# Autodesk Inventor assembly: TelescopingArm_MIR1
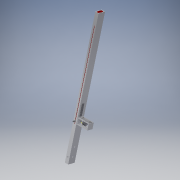
[picture p0: Inventor's stored thumbnail of the model, 180x180]
Saved by Autodesk Inventor 2016 SP1 (Build 200210100, 210)
## iProperties
Created: 2016-01-26
Part Number: TelescopingArm_MIR1
Document SubType Name: Assembly
Designer: steele
Mass: 2430.38 g
Surface Area: 5620.49 cm^2
Volume: 865.213 cm^3
Density: 2.80899 g/cm^3
Author: steele
## Documents named in this file (7)
- C:\snobotics\CAD-Development\robSteele\SnoBotics2016\TelescopeArm\TelescopingArm_MIR1.iam
- C:\snobotics\CAD-Development\robSteele\SnoBotics2016\TelescopeArm\OuterTube_MIR2.ipt
- C:\snobotics\CAD-Development\robSteele\SnoBotics2016\TelescopeArm\InnerTube_MIR2.ipt
- C:\snobotics\CAD-Development\robSteele\SnoBotics2016\2016-01-31-Lift\InnerTubeStopPost_MIR.ipt
- C:\snobotics\CAD-Development\robSteele\SnoBotics2016\2016-02-17-StopMechanism\StopMechanismAssembly_MIR.iam
- C:\snobotics\CAD-Development\robSteele\SnoBotics2016\AM Parts\AM 2488 CIM bracket_MIR7.ipt
- C:\snobotics\CAD-Development\robSteele\SnoBotics2016\AM Parts\MOT_CIM-Motor_217-2000_MIR7_MIR.iam
## Components (6 placed, 6 different names)
1. OuterTube_MIR2:1 — Mate:2, Mate:1, Insert:2, Flush:1, Flush:3, Flush:2, Mate:3
2. InnerTube_MIR2:1 — Mate:2, Mate:1, Insert:1
3. InnerTubeStopPost_MIR:1 — Insert:1
4. StopMechanismAssembly_MIR:1 [sub-assembly] — Insert:2, Flush:1
5. AM 2488 CIM bracket_MIR7:1 — Flush:3, Flush:2, Mate:3, Insert:3
6. MOT_CIM-Motor_217-2000_MIR7_MIR:1 [sub-assembly] — Insert:3
## Relationships (9: Flush 5, Insert 3, Mate 1)
- Mate:2 [Flush]: OuterTube_MIR2:1 ↔ InnerTube_MIR2:1
- Mate:1 [Flush]: OuterTube_MIR2:1 ↔ InnerTube_MIR2:1
- Insert:1 (31.75 mm): InnerTube_MIR2:1 ↔ InnerTubeStopPost_MIR:1
- Insert:2 (3.683 mm): OuterTube_MIR2:1 ↔ StopMechanismAssembly_MIR:1
- Flush:1: OuterTube_MIR2:1 ↔ StopMechanismAssembly_MIR:1
- Flush:3 (-127 mm): OuterTube_MIR2:1 ↔ AM 2488 CIM bracket_MIR7:1
- Flush:2: OuterTube_MIR2:1 ↔ AM 2488 CIM bracket_MIR7:1
- Mate:3: OuterTube_MIR2:1 ↔ AM 2488 CIM bracket_MIR7:1
- Insert:3: AM 2488 CIM bracket_MIR7:1 ↔ MOT_CIM-Motor_217-2000_MIR7_MIR:1
